# Autodesk Inventor assembly: drive
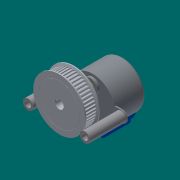
[picture p0: Inventor's stored thumbnail of the model, 180x180]
Saved by Autodesk Inventor 2016 (Build 200138000, 138)
## iProperties
Created: 2015-10-05
Part Number: drive
Document SubType Name: Assembly
Designer: Sawaiz
Author: Sawaiz
## Documents named in this file (4)
- C:\Users\sawai\OneDrive\projects\splitFlapDisplay\drive\drive.iam
- C:\Users\sawai\OneDrive\projects\splitFlapDisplay\electronics\stepperMotor.ipt
- C:\Users\sawai\OneDrive\projects\splitFlapDisplay\drive\gt250Tooth.ipt
- C:\Users\sawai\OneDrive\projects\splitFlapDisplay\drive\motorSpacer.ipt
## Components (4 placed, 3 different names)
1. stepperMotor:1 — Mate:1, Mate:2, Mate:3, Mate:4, Mate:5, Mate:6
2. gt250Tooth:1 — Mate:1, Mate:2
3. motorSpacer:1 — Mate:3, Mate:6
4. motorSpacer:2 — Mate:4, Mate:5
## Relationships (6: Mate 6)
- Mate:1: stepperMotor:1 ↔ gt250Tooth:1
- Mate:2: stepperMotor:1 ↔ gt250Tooth:1
- Mate:3: stepperMotor:1 ↔ motorSpacer:1
- Mate:4: stepperMotor:1 ↔ motorSpacer:2
- Mate:5: stepperMotor:1 ↔ motorSpacer:2
- Mate:6: stepperMotor:1 ↔ motorSpacer:1
